# Autodesk Inventor assembly: full
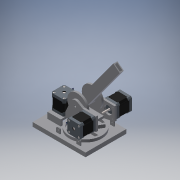
[picture p0: Inventor's stored thumbnail of the model, 180x180]
Saved by Autodesk Inventor 2019 (Build 230136000, 136)
## iProperties
Created: 2019-05-02
Part Number: full
Document SubType Name: Assembly
Designer: Nathan
Author: Nathan
## Documents named in this file (5)
- C:\Users\Nathan\workspace\fbd-brachium\cad\full.iam
- C:\Users\Nathan\workspace\fbd-brachium\cad\shoulder.ipt
- C:\Users\Nathan\workspace\fbd-brachium\cad\Nema17.ipt
- C:\Users\Nathan\workspace\fbd-brachium\cad\arm_proximal.ipt
- C:\Users\Nathan\workspace\fbd-brachium\cad\base.ipt
## Components (6 placed, 4 different names)
1. shoulder:1 — Insert:1, Insert:2, Insert:3, Insert:4, Insert:5, Insert:9
2. Nema17:1 — Insert:1, Insert:2
3. Nema17:2 — Insert:3, Insert:4
4. arm_proximal:1 — Insert:5
5. base:1 — Insert:7, Insert:8, Insert:9
6. Nema17:3 — Insert:7, Insert:8
## Relationships (8: Insert 8)
- Insert:1: shoulder:1 ↔ Nema17:1
- Insert:2: shoulder:1 ↔ Nema17:1
- Insert:3: shoulder:1 ↔ Nema17:2
- Insert:4: shoulder:1 ↔ Nema17:2
- Insert:5: shoulder:1 ↔ arm_proximal:1
- Insert:7: base:1 ↔ Nema17:3
- Insert:8: base:1 ↔ Nema17:3
- Insert:9: shoulder:1 ↔ base:1
